# Autodesk Inventor assembly: Final Robot
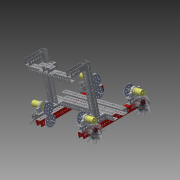
[picture p0: Inventor's stored thumbnail of the model, 180x180]
Saved by Autodesk Inventor 2015 (Build 190159000, 159)
## iProperties
Created: 2015-02-14
Part Number: Final Robot
Document SubType Name: Assembly
Designer: Bhaskar
Author: Bhaskar
## Documents named in this file (4)
- C:\Users\Bhaskar\Desktop\RoboCAD\CAD\Final Robot.iam
- C:\Users\Bhaskar\Desktop\RoboCAD\CAD\base.iam
- C:\Users\Bhaskar\Desktop\RoboCAD\CAD\RobotSpine.iam
- C:\Users\Bhaskar\Desktop\RoboCAD\CAD\Imported Components\L Bracket\Assembly3.iam
## Components (4 placed, 3 different names)
1. base:1 [sub-assembly] — Insert:1, Angle:1, Insert:2, Angle:2
2. RobotSpine:1 [sub-assembly] — Insert:3, Insert:4
3. Assembly3:1 [sub-assembly] — Insert:1, Angle:1, Insert:3
4. Assembly3:2 [sub-assembly] — Insert:2, Angle:2, Insert:4
## Relationships (6: Insert 4, Angle 2)
- Insert:1: base:1 ↔ Assembly3:1
- Angle:1 (0 deg): base:1 ↔ Assembly3:1
- Insert:2: base:1 ↔ Assembly3:2
- Angle:2 (0 deg): base:1 ↔ Assembly3:2
- Insert:3: RobotSpine:1 ↔ Assembly3:1
- Insert:4: RobotSpine:1 ↔ Assembly3:2
